# Autodesk Inventor assembly: BallSensorUnit
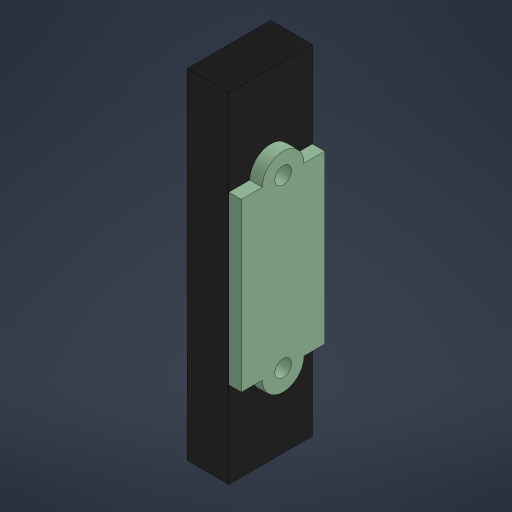
[picture p0: Inventor's stored thumbnail of the model, 512x512]
Saved by Autodesk Inventor 2024.2 (Build 282272000, 272)
## iProperties
Created: 2023-12-28
Part Number: BallSensorUnit
Document SubType Name: Assembly
Designer: Hanaoka
Author: Hanaoka
## Documents named in this file (3)
- G:\共有ドライブ\reRo\05_個人\hanaoka\inventor\BallSensorUnit\BallSensorUnit.iam
- G:\共有ドライブ\reRo\05_個人\hanaoka\inventor\BallSensorUnit\BallSensor_Mount.ipt
- G:\共有ドライブ\reRo\05_個人\hanaoka\inventor\BallSensorUnit\BallSensor_PCB.ipt
## Components (2 placed, 2 different names)
1. BallSensor_Mount:1 — フラッシュ:1
2. BallSensor_PCB:1 — フラッシュ:1
## Relationships (1: Flush 1)
- フラッシュ:1 [Flush]: BallSensor_Mount:1 ↔ BallSensor_PCB:1
